# Autodesk Inventor assembly: Gobilda bevel gears + 8mm REX hyper hub_MIR
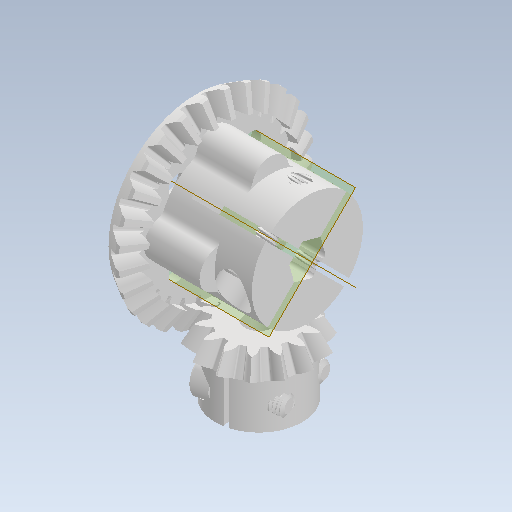
[picture p0: Inventor's stored thumbnail of the model, 512x512]
Saved by Autodesk Inventor 2020 (Build 240168000, 168)
## iProperties
Created: 2020-02-29
Part Number: Gobilda bevel gears + 8mm REX hyper hub_MIR
Document SubType Name: Assembly
Designer: jackm
Author: ball
## Documents named in this file (4)
- D:\FTC8863\2019 Robot\Generic Parts\Gobilda bevel gears + 8mm REX hyper hub_MIR.iam
- D:\FTC8863\GoBilda\3204 Parts\3204-0002-0001 assembly_MIR.iam
- D:\FTC8863\GoBilda\1310 Parts\1310-0016-4008 assembly_MIR.ipt
- D:\FTC8863\StepLibraries\Screws\M4 x 12 SOCKET HEAD CAP SCREW_MIR.ipt
## Components (6 placed, 3 different names)
1. 3204-0002-0001 assembly_MIR:1 [sub-assembly] — Mate:4, Mate:3, Mate:2, Mate:1, Mate:11, Mate:5, Mate:12, Mate:6, Mate:10, Mate:7, Mate:9, Mate:8
2. 1310-0016-4008 assembly_MIR:1 — Mate:4, Mate:3, Mate:2, Mate:1
3. M4 x 12 SOCKET HEAD CAP SCREW_MIR:1 — Mate:11, Mate:5
4. M4 x 12 SOCKET HEAD CAP SCREW_MIR:2 — Mate:12, Mate:6
5. M4 x 12 SOCKET HEAD CAP SCREW_MIR:3 — Mate:10, Mate:7
6. M4 x 12 SOCKET HEAD CAP SCREW_MIR:4 — Mate:9, Mate:8
## Relationships (12: Mate 12)
- Mate:4: 3204-0002-0001 assembly_MIR:1 ↔ 1310-0016-4008 assembly_MIR:1
- Mate:3: 3204-0002-0001 assembly_MIR:1 ↔ 1310-0016-4008 assembly_MIR:1
- Mate:2: 3204-0002-0001 assembly_MIR:1 ↔ 1310-0016-4008 assembly_MIR:1
- Mate:1: 3204-0002-0001 assembly_MIR:1 ↔ 1310-0016-4008 assembly_MIR:1
- Mate:11: 3204-0002-0001 assembly_MIR:1 ↔ M4 x 12 SOCKET HEAD CAP SCREW_MIR:1
- Mate:5: 3204-0002-0001 assembly_MIR:1 ↔ M4 x 12 SOCKET HEAD CAP SCREW_MIR:1
- Mate:12: 3204-0002-0001 assembly_MIR:1 ↔ M4 x 12 SOCKET HEAD CAP SCREW_MIR:2
- Mate:6: 3204-0002-0001 assembly_MIR:1 ↔ M4 x 12 SOCKET HEAD CAP SCREW_MIR:2
- Mate:10: 3204-0002-0001 assembly_MIR:1 ↔ M4 x 12 SOCKET HEAD CAP SCREW_MIR:3
- Mate:7: 3204-0002-0001 assembly_MIR:1 ↔ M4 x 12 SOCKET HEAD CAP SCREW_MIR:3
- Mate:9: 3204-0002-0001 assembly_MIR:1 ↔ M4 x 12 SOCKET HEAD CAP SCREW_MIR:4
- Mate:8: 3204-0002-0001 assembly_MIR:1 ↔ M4 x 12 SOCKET HEAD CAP SCREW_MIR:4
